# Autodesk Inventor assembly: Health_module
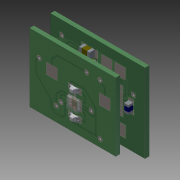
[picture p0: Inventor's stored thumbnail of the model, 180x180]
Saved by Autodesk Inventor 2013 (Build 170138000, 138)
## iProperties
Created: 2015-07-04
Part Number: Health_module
Document SubType Name: Assembly
Designer: terg
Author: terg
## Documents named in this file (3)
- C:\Users\terg\Projects\ModularElectronics\3D_models\Health_module\Health_module.iam
- C:\Users\terg\Projects\ModularElectronics\3D_models\Health_module\Health_module_ucBoard.iam
- C:\Users\terg\Projects\ModularElectronics\3D_models\Health_module\Health_module_contactBoard.iam
## Components (2 placed, 2 different names)
1. Health_module_ucBoard:1 [sub-assembly] — Zestawiający:1, Zestawiający:2, Zestawiający:3
2. Health_module_contactBoard:1 [sub-assembly] — Zestawiający:1, Zestawiający:2, Zestawiający:3
## Relationships (3: Mate 3)
- Zestawiający:1 [Mate] (3 mm): Health_module_ucBoard:1 ↔ Health_module_contactBoard:1
- Zestawiający:2 [Mate] (-4.766 mm): Health_module_ucBoard:1 ↔ Health_module_contactBoard:1
- Zestawiający:3 [Mate] (-2.525 mm): Health_module_ucBoard:1 ↔ Health_module_contactBoard:1
